# Autodesk Inventor assembly: Assembly Proximity V3
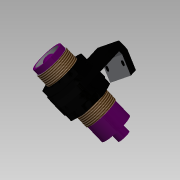
[picture p0: Inventor's stored thumbnail of the model, 180x180]
Saved by Autodesk Inventor 2015 SP1 (Build 190203100, 203)
## iProperties
Created: 2015-01-28
Part Number: Assembly Proximity V3
Document SubType Name: Assembly
Designer: Rafi Kurnia Putra
Author: Rafi Kurnia Putra
## Documents named in this file (4)
- D:\Dropbox\krpai berkaki trui 2015\ROBUSTA\MEKANIK\ROBUSTA\Assembly Proximity V3.iam
- D:\Dropbox\krpai berkaki trui 2015\ROBUSTA\MEKANIK\ROBUSTA\Proximity.ipt
- D:\Dropbox\krpai berkaki trui 2015\ROBUSTA\MEKANIK\ROBUSTA\Proximity Gear.ipt
- D:\Dropbox\krpai berkaki trui 2015\ROBUSTA\MEKANIK\ROBUSTA\Dudukan Proximity V3.ipt
## Components (4 placed, 3 different names)
1. Proximity:1 — Rigid:1, Rigid:2, Mate:2
2. Proximity Gear:1 — Rigid:2
3. Proximity Gear:2 — Rigid:1, Mate:1
4. Dudukan Proximity V3:1 — Mate:1, Mate:2
## Relationships (4: WeldJoint 2, Mate 2)
- Rigid:1 [WeldJoint] (-15 mm): Proximity:1 ↔ Proximity Gear:2
- Rigid:2 [WeldJoint] (-15 mm): Proximity:1 ↔ Proximity Gear:1
- Mate:1: Proximity Gear:2 ↔ Dudukan Proximity V3:1
- Mate:2: Proximity:1 ↔ Dudukan Proximity V3:1
